# Autodesk Inventor assembly: Thumb Assem
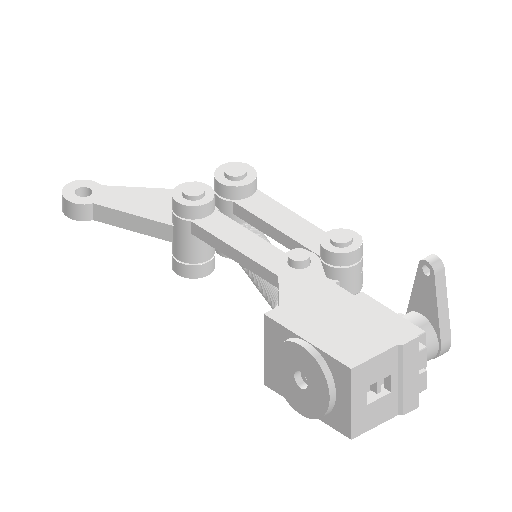
[picture p0: Inventor's stored thumbnail of the model, 512x512]
Saved by Autodesk Inventor 2025.1 (Build 291241020, 241B)
## iProperties
Created: 2024-12-05
Part Number: Thumb Assem
Document SubType Name: Assembly
Designer: ALEXANDERNICHOLS
Author: ALEXANDERNICHOLS
## Documents named in this file (12)
- D:\CAD\Inventor\Bio Kettering Hand\Liv Mas 1.0\Thumb Assem.iam
- D:\CAD\Inventor\Bio Kettering Hand\Liv Mas 1.0\Arm 1.ipt
- D:\CAD\Inventor\Bio Kettering Hand\Liv Mas 1.0\Arm 2.ipt
- D:\CAD\Inventor\Bio Kettering Hand\Liv Mas 1.0\Arm 3.ipt
- D:\CAD\Inventor\Bio Kettering Hand\Liv Mas 1.0\Servo Spinner.ipt
- D:\CAD\Inventor\Bio Kettering Hand\Liv Mas 1.0\Washer.ipt
- D:\CAD\Inventor\Bio Kettering Hand\Liv Mas 1.0\Servo.ipt
- D:\CAD\Inventor\Bio Kettering Hand\Liv Mas 1.0\Spring Holder.ipt
- D:\CAD\Inventor\Bio Kettering Hand\Liv Mas 1.0\Screw PROP.ipt
- D:\CAD\Inventor\Bio Kettering Hand\Liv Mas 1.0\Servo Base Thumb.ipt
- D:\CAD\Inventor\Bio Kettering Hand\Liv Mas 1.0\Spring PROP.ipt
- D:\CAD\Inventor\Bio Kettering Hand\Liv Mas 1.0\Tip Arm 1.ipt
## Components (21 placed, 11 different names)
1. Arm 1:1 — Rotational:2, Rotational:3, Rotational:11, Rotational:14
2. Arm 2:1 — Rotational:11, Rotational:18, Rotational:20, Rotational:26
3. Arm 3:1 — Rotational:2, Rotational:19, Rotational:24
4. Servo Spinner:1 — Rotational:13
5. Washer:1 — Rotational:15
6. Servo:1 — Rotational:13, Mate:1, Mate:2, Mate:3
7. Spring Holder:1 — Rotational:16, Mate:9, Flush:2, Mate:10
8. Spring Holder:2 — Rotational:3, Mate:11
9. Spring Holder:3 — Rotational:14, Rotational:15
10. Washer:2 — Rotational:16, Mate:6, Flush:1
11. Washer:3 — Mate:8, Flush:1
12. Washer:4 — Rotational:18, Rotational:21
13. Washer:5 — Rotational:19, Rotational:23
14. Washer:6 — Rotational:20, Rotational:22
15. Screw PROP:1 — Rotational:21
16. Screw PROP:2 — Rotational:22, Mate:6
17. Screw PROP:3 — Rotational:23, Mate:7, Mate:8
18. Screw PROP:4 — Rotational:25
19. Servo Base Thumb:1 — Rotational:24, Rotational:25, Mate:1, Mate:2, Mate:3
20. Tip Arm 1:1 — Rotational:26, Mate:7, Mate:9
21. Spring PROP:1 — Flush:2, Mate:10, Mate:11
## Relationships (27: RevoluteJoint 16, Mate 9, Flush 2)
- Rotational:2 [RevoluteJoint]: Arm 1:1 ↔ Arm 3:1
- Rotational:3 [RevoluteJoint]: Arm 1:1 ↔ Spring Holder:2
- Rotational:11 [RevoluteJoint]: Arm 1:1 ↔ Arm 2:1
- Rotational:13 [RevoluteJoint]: Servo Spinner:1 ↔ Servo:1
- Rotational:14 [RevoluteJoint]: Arm 1:1 ↔ Spring Holder:3
- Rotational:15 [RevoluteJoint] (-0.508 mm): Washer:1 ↔ Spring Holder:3
- Rotational:16 [RevoluteJoint] (-0.508 mm): Spring Holder:1 ↔ Washer:2
- Rotational:18 [RevoluteJoint] (0.508 mm): Arm 2:1 ↔ Washer:4
- Rotational:19 [RevoluteJoint] (0.508 mm): Arm 3:1 ↔ Washer:5
- Rotational:20 [RevoluteJoint] (0.508 mm): Arm 2:1 ↔ Washer:6
- Rotational:21 [RevoluteJoint]: Washer:4 ↔ Screw PROP:1
- Rotational:22 [RevoluteJoint]: Washer:6 ↔ Screw PROP:2
- Rotational:23 [RevoluteJoint]: Washer:5 ↔ Screw PROP:3
- Rotational:24 [RevoluteJoint]: Arm 3:1 ↔ Servo Base Thumb:1
- Rotational:25 [RevoluteJoint]: Screw PROP:4 ↔ Servo Base Thumb:1
- Mate:1: Servo:1 ↔ Servo Base Thumb:1
- Mate:2: Servo:1 ↔ Servo Base Thumb:1
- Mate:3: Servo:1 ↔ Servo Base Thumb:1
- Rotational:26 [RevoluteJoint]: Arm 2:1 ↔ Tip Arm 1:1
- Mate:6: Washer:2 ↔ Screw PROP:2
- Mate:7: Screw PROP:3 ↔ Tip Arm 1:1
- Mate:8: Washer:3 ↔ Screw PROP:3
- Flush:1: Washer:2 ↔ Washer:3
- Mate:9: Spring Holder:1 ↔ Tip Arm 1:1
- Flush:2: Spring Holder:1 ↔ Spring PROP:1
- Mate:10: Spring Holder:1 ↔ Spring PROP:1
- Mate:11: Spring Holder:2 ↔ Spring PROP:1
